# Autodesk Inventor assembly: 40-J4
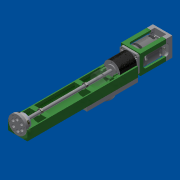
[picture p0: Inventor's stored thumbnail of the model, 180x180]
Saved by Autodesk Inventor 2018 (Build 220112000, 112)
## iProperties
Created: 2020-06-07
Part Number: 40-J4
Document SubType Name: Assembly
Designer: Bunny320
Author: Bunny320
## Documents named in this file (10)
- C:\Users\Bunny320\Desktop\sechs\4-CAD\40-J4.iam
- C:\Users\Bunny320\Desktop\sechs\4-CAD\motor unit 2820.iam
- C:\Users\Bunny320\Desktop\sechs\4-CAD\401-flange.ipt
- C:\Users\Bunny320\Desktop\sechs\4-CAD\402-gearbox-housing.ipt
- C:\Users\Bunny320\Desktop\sechs\4-CAD\403-coupler dummy.ipt
- C:\Users\Bunny320\Desktop\sechs\4-CAD\404-shaft.ipt
- C:\Users\Bunny320\Desktop\sechs\4-CAD\standardParts\Pololu mounting hub\pololu-universal-aluminum-mounting-hub-for-6mm-shaft-m3-holes.ipt
- C:\Users\Bunny320\Desktop\sechs\4-CAD\standardParts\61705-2RZ\W 61705-2RZ.iam
- C:\Users\Bunny320\Desktop\sechs\4-CAD\405-output disk.ipt
- C:\Users\Bunny320\Desktop\sechs\4-CAD\standardParts\W 627_6-2Z\W 627_6-2Z.iam
## Components (10 placed, 9 different names)
1. motor unit 2820:1 [sub-assembly] — Flush:1, Flush:2, Flush:3, Mate:1, Mate:2, Mate:3, Mate:5, Mate:12
2. 401-flange:1 — Mate:1, Flush:5, Flush:6, Mate:17
3. 402-gearbox-housing:1 — Mate:2, Mate:3, Flush:5, Flush:6, Mate:15, Mate:16
4. 403-coupler dummy:1 — Mate:5, Mate:6
5. 404-shaft:1 — Mate:6, Mate:7, Flush:7, Mate:12, Mate:13, Mate:14
6. pololu-universal-aluminum-mounting-hub-for-6mm-shaft-m3-holes:1 — Mate:7, Flush:7, Mate:10
7. W 61705-2RZ:1 [sub-assembly] — Mate:10, Mate:11, Mate:18
8. 405-output disk:1 — Mate:11, Mate:17, Mate:18
9. W 627_6-2Z:1 [sub-assembly] — Mate:13, Mate:15
10. W 627_6-2Z:2 [sub-assembly] — Mate:14, Mate:16
## Relationships (21: Mate 15, Flush 6)
- Flush:1: motor unit 2820:1
- Flush:2: motor unit 2820:1
- Flush:3: motor unit 2820:1
- Mate:1: motor unit 2820:1 ↔ 401-flange:1
- Mate:2: motor unit 2820:1 ↔ 402-gearbox-housing:1
- Mate:3: motor unit 2820:1 ↔ 402-gearbox-housing:1
- Flush:5: 401-flange:1 ↔ 402-gearbox-housing:1
- Flush:6: 401-flange:1 ↔ 402-gearbox-housing:1
- Mate:5: motor unit 2820:1 ↔ 403-coupler dummy:1
- Mate:6: 403-coupler dummy:1 ↔ 404-shaft:1
- Mate:7: 404-shaft:1 ↔ pololu-universal-aluminum-mounting-hub-for-6mm-shaft-m3-holes:1
- Flush:7: 404-shaft:1 ↔ pololu-universal-aluminum-mounting-hub-for-6mm-shaft-m3-holes:1
- Mate:10: pololu-universal-aluminum-mounting-hub-for-6mm-shaft-m3-holes:1 ↔ W 61705-2RZ:1
- Mate:11: W 61705-2RZ:1 ↔ 405-output disk:1
- Mate:12 (2 mm): motor unit 2820:1 ↔ 404-shaft:1
- Mate:13: 404-shaft:1 ↔ W 627_6-2Z:1
- Mate:14: 404-shaft:1 ↔ W 627_6-2Z:2
- Mate:15: 402-gearbox-housing:1 ↔ W 627_6-2Z:1
- Mate:16: 402-gearbox-housing:1 ↔ W 627_6-2Z:2
- Mate:17 (-168 mm): 401-flange:1 ↔ 405-output disk:1
- Mate:18: W 61705-2RZ:1 ↔ 405-output disk:1
